# Autodesk Inventor assembly: iris_mecanico
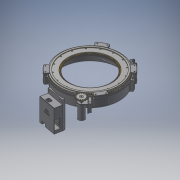
[picture p0: Inventor's stored thumbnail of the model, 180x180]
Saved by Autodesk Inventor 2019 (Build 230136000, 136)
## iProperties
Created: 2020-08-08
Part Number: iris_mecanico
Document SubType Name: Assembly
Designer: Hugo Albarracin
Author: Hugo Albarracin
## Documents named in this file (14)
- C:\Users\Hugo Albarracin\OneDrive - Escuela Superior Politécnica del Litoral\U - UPM ELECTROMECANICA\14. TFM\iris_mecanico\iris_mecanico.iam
- C:\Users\Hugo Albarracin\OneDrive - Escuela Superior Politécnica del Litoral\U - UPM ELECTROMECANICA\14. TFM\iris_mecanico\Alabe_pivote.ipt
- C:\Users\Hugo Albarracin\OneDrive - Escuela Superior Politécnica del Litoral\U - UPM ELECTROMECANICA\14. TFM\iris_mecanico\Alabes.ipt
- C:\Users\Hugo Albarracin\OneDrive - Escuela Superior Politécnica del Litoral\U - UPM ELECTROMECANICA\14. TFM\iris_mecanico\Anillo_inferior.ipt
- C:\Users\Hugo Albarracin\OneDrive - Escuela Superior Politécnica del Litoral\U - UPM ELECTROMECANICA\14. TFM\iris_mecanico\Collarin_base.ipt
- C:\Users\Hugo Albarracin\OneDrive - Escuela Superior Politécnica del Litoral\U - UPM ELECTROMECANICA\14. TFM\iris_mecanico\Anillo_superior.ipt
- C:\Users\Hugo Albarracin\OneDrive - Escuela Superior Politécnica del Litoral\U - UPM ELECTROMECANICA\14. TFM\iris_mecanico\Rueda_motriz.ipt
- C:\Users\Hugo Albarracin\OneDrive - Escuela Superior Politécnica del Litoral\U - UPM ELECTROMECANICA\14. TFM\iris_mecanico\sistema_motriz\sistema_motriz.iam
- C:\Users\Hugo Albarracin\OneDrive - Escuela Superior Politécnica del Litoral\U - UPM ELECTROMECANICA\14. TFM\iris_mecanico\sistema_motriz\conexion_motor_rueda.ipt
- C:\Users\Hugo Albarracin\OneDrive - Escuela Superior Politécnica del Litoral\U - UPM ELECTROMECANICA\14. TFM\iris_mecanico\soporte fotocelda.ipt
- C:\Users\Hugo Albarracin\OneDrive - Escuela Superior Politécnica del Litoral\U - UPM ELECTROMECANICA\14. TFM\iris_mecanico\Soporte placa.iam
- C:\Users\Hugo Albarracin\OneDrive - Escuela Superior Politécnica del Litoral\U - UPM ELECTROMECANICA\14. TFM\iris_mecanico\accesorios separador 2.2.ipt
- C:\Users\Hugo Albarracin\OneDrive - Escuela Superior Politécnica del Litoral\U - UPM ELECTROMECANICA\14. TFM\iris_mecanico\accesorios separador 2.3.ipt
- C:\Users\Hugo Albarracin\OneDrive - Escuela Superior Politécnica del Litoral\U - UPM ELECTROMECANICA\14. TFM\iris_mecanico\iris_mecanico_parametrizacion.xlsx
## Components (60 placed, 12 different names)
1. Anillo_inferior:1 — Mate:4, Mate:9, Mate:10, Mate:11, Mate:18, Mate:40
2. Collarin_base:1 — Mate:1, Mate:2, Mate:3, Mate:4, Mate:9, Mate:10, Flush:1, Mate:12, Flush:2, Mate:23, Mate:24, Mate:25, Mate:26, Mate:27, Mate:28, Mate:30, Mate:31, Mate:34, Mate:35, Mate:37, Mate:39
3. Spur Gear2:1 — Mate:11, Mate:19, Mate:20, Mate:21, Rotation:1, Mate:29, Mate:32, Mate:33, Mate:38
4. sistema_motriz:1 [sub-assembly] — Flush:1, Mate:12, Flush:2, Mate:13, Mate:16
5. conexion_motor_rueda:1 — Mate:13, Flush:3, Mate:14, Mate:15, Mate:16
6. Spur Gear1:2 — Flush:3, Mate:14, Mate:15, Rotation:1
7. soporte fotocelda:1 — Mate:23, Mate:24
8. Soporte placa:1 [sub-assembly] — Mate:25, Mate:26
9. accesorios separador 2.2:1 — Mate:33, Mate:34, Mate:35
10. accesorios separador 2.3:1 — Mate:27, Mate:28, Mate:29
11. accesorios separador 2.2:2 — Mate:37, Mate:38, Mate:39
12. accesorios separador 2.3:2 — Mate:30, Mate:31, Mate:32
13. Alabes:1 — Mate:5, Mate:6, Mate:7, Mate:8, Mate:18
14. Alabe_pivote:1 — Mate:5, Mate:6, Mate:20, Mate:40
15. Alabe_pivote:2 — Mate:7, Mate:8, Mate:19, Mate:21
16. Alabes:2
17. Alabe_pivote:3
18. Alabe_pivote:4
19. Alabes:3
20. Alabe_pivote:5
21. Alabe_pivote:6
22. Alabes:4
23. Alabe_pivote:7
24. Alabe_pivote:8
25. Alabes:5
26. Alabe_pivote:9
27. Alabe_pivote:10
28. Alabes:6
29. Alabe_pivote:11
30. Alabe_pivote:12
31. Alabes:7
32. Alabe_pivote:13
33. Alabe_pivote:14
34. Alabes:8
35. Alabe_pivote:15
36. Alabe_pivote:16
37. Alabes:9
38. Alabe_pivote:17
39. Alabe_pivote:18
40. Alabes:10
41. Alabe_pivote:19
42. Alabe_pivote:20
43. Alabes:11
44. Alabe_pivote:21
45. Alabe_pivote:22
46. Alabes:12
47. Alabe_pivote:23
48. Alabe_pivote:24
49. Alabes:13
50. Alabe_pivote:25
51. Alabe_pivote:26
52. Alabes:14
53. Alabe_pivote:27
54. Alabe_pivote:28
55. Alabes:15
56. Alabe_pivote:29
57. Alabe_pivote:30
58. Alabes:16
59. Alabe_pivote:31
60. Alabe_pivote:32
## Component patterns: (16 elements, first: Alabes:1 + Alabe_pivote:1 + Alabe_pivote:2)
## Relationships (41: Mate 37, Flush 3, RelateRotation 1)
- Mate:1: Collarin_base:1
- Mate:2: Collarin_base:1
- Mate:3: Collarin_base:1
- Mate:4: Anillo_inferior:1 ↔ Collarin_base:1
- Mate:5: Alabes:1 ↔ Alabe_pivote:1
- Mate:6: Alabes:1 ↔ Alabe_pivote:1
- Mate:7: Alabes:1 ↔ Alabe_pivote:2
- Mate:8: Alabes:1 ↔ Alabe_pivote:2
- Mate:9: Anillo_inferior:1 ↔ Collarin_base:1
- Mate:10: Anillo_inferior:1 ↔ Collarin_base:1
- Mate:11: Anillo_inferior:1 ↔ Spur Gear2:1
- Flush:1: Collarin_base:1 ↔ sistema_motriz:1
- Mate:12: Collarin_base:1 ↔ sistema_motriz:1
- Flush:2 (6 mm): Collarin_base:1 ↔ sistema_motriz:1
- Mate:13: sistema_motriz:1 ↔ conexion_motor_rueda:1
- Flush:3: conexion_motor_rueda:1 ↔ Spur Gear1:2
- Mate:14: conexion_motor_rueda:1 ↔ Spur Gear1:2
- Mate:15: conexion_motor_rueda:1 ↔ Spur Gear1:2
- Mate:16: sistema_motriz:1 ↔ conexion_motor_rueda:1
- Mate:18: Anillo_inferior:1 ↔ Alabes:1
- Mate:19: Spur Gear2:1 ↔ Alabe_pivote:2
- Mate:20: Spur Gear2:1 ↔ Alabe_pivote:1
- Mate:21: Spur Gear2:1 ↔ Alabe_pivote:2
- Rotation:1 [RelateRotation] (7.0588 ul): Spur Gear2:1 ↔ Spur Gear1:2
- Mate:23: Collarin_base:1 ↔ soporte fotocelda:1
- Mate:24: Collarin_base:1 ↔ soporte fotocelda:1
- Mate:25: Collarin_base:1 ↔ Soporte placa:1
- Mate:26: Collarin_base:1 ↔ Soporte placa:1
- Mate:27: Collarin_base:1 ↔ accesorios separador 2.3:1
- Mate:28: Collarin_base:1 ↔ accesorios separador 2.3:1
- Mate:29: Spur Gear2:1 ↔ accesorios separador 2.3:1
- Mate:30: Collarin_base:1 ↔ accesorios separador 2.3:2
- Mate:31: Collarin_base:1 ↔ accesorios separador 2.3:2
- Mate:32: Spur Gear2:1 ↔ accesorios separador 2.3:2
- Mate:33: Spur Gear2:1 ↔ accesorios separador 2.2:1
- Mate:34: Collarin_base:1 ↔ accesorios separador 2.2:1
- Mate:35: Collarin_base:1 ↔ accesorios separador 2.2:1
- Mate:37: Collarin_base:1 ↔ accesorios separador 2.2:2
- Mate:38: Spur Gear2:1 ↔ accesorios separador 2.2:2
- Mate:39: Collarin_base:1 ↔ accesorios separador 2.2:2
- Mate:40: Anillo_inferior:1 ↔ Alabe_pivote:1
## Named parameters: num_alabes = 16, angulo_alabe = 130 deg, ancho_disco = 30 mm, diametro_max = 240 mm, diametro_tubo = 232 mm, ancho_estructura = 280 mm, desfase_a_pin_superior = 12 mm, desfase_a_pin_inferior = 10 mm, desfase_b_pin_inferior = 8 mm, desfase_b_pin_superior = 0 mm, diametro_pin = 10 mm, diametro_max_soporte = 248 mm, num_z = 120
